# Autodesk Inventor assembly: XM430-Working-Shaft
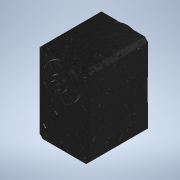
[picture p0: Inventor's stored thumbnail of the model, 180x180]
Saved by Autodesk Inventor 2021 (Build 250183000, 183)
## iProperties
Created: 2022-05-12
Part Number: XM430-Working-Shaft
Document SubType Name: Assembly
Designer: alyn649
Sending System: Autodesk Inventor 2022
Preprocessor: ST-DEVELOPER v18.1
Title: G:\Uni\Part4Project\p4p\CAD\Step\XM430-Working-Shaft.stp
Author: User
Revision Number: 4LAST_VERSION
## Documents named in this file (6)
- \\files.auckland.ac.nz\myhome\Documents\GitHub\hand\XM430 Motor\XM430-Working-Shaft.iam
- \\files.auckland.ac.nz\myhome\Documents\GitHub\hand\XM430 Motor\DUMMY_DC12.ipt
- \\files.auckland.ac.nz\myhome\Documents\GitHub\hand\XM430 Motor\WBH_M2_5X12.ipt
- \\files.auckland.ac.nz\myhome\Documents\GitHub\hand\XM430 Motor\DC12_A01_SPACER_RING_1.ipt
- \\files.auckland.ac.nz\myhome\Documents\GitHub\hand\XM430 Motor\DC12_A01_CVR_CABLE_5.ipt
- \\files.auckland.ac.nz\myhome\Documents\GitHub\hand\XM430 Motor\XM430-Shaft.ipt
## Components (19 placed, 19 different names)
1. 36 — Rotational:1, Rotational:2
2. 37
3. 38
4. 39
5. 40
6. 41
7. 42
8. 43 — Rotational:2
9. 44
10. 45
11. 46
12. 47
13. 48
14. 49
15. 50
16. 51
17. 52
18. 53
19. XM430-Shaft:1 — Rotational:1
## Relationships (2: RevoluteJoint 2)
- Rotational:1 [RevoluteJoint]: 36 ↔ XM430-Shaft:1
- Rotational:2 [RevoluteJoint]: 36 ↔ 43
